# Autodesk Inventor assembly: ASTRA
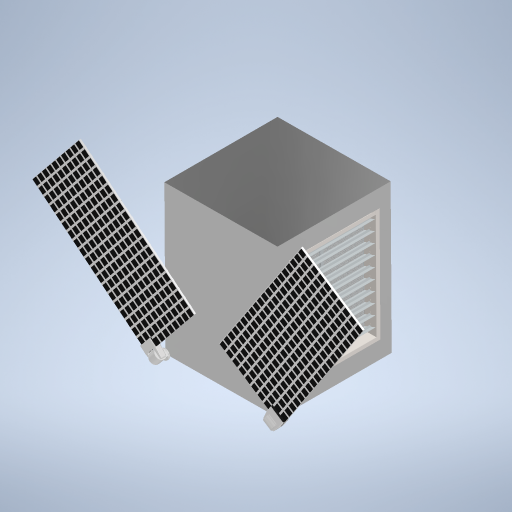
[picture p0: Inventor's stored thumbnail of the model, 512x512]
Saved by Autodesk Inventor 2023.2 (Build 272271030, 271C)
## iProperties
Created: 2023-04-10
Part Number: ASTRA
Document SubType Name: Assembly
Designer: ckeer
Author: ckeer
## Documents named in this file (5)
- F:\Github\School\Prelim\CAD\ASTRA.iam
- F:\Github\School\Prelim\CAD\Solar Panel.ipt
- F:\Github\School\Prelim\CAD\ASTRA_Body.ipt
- F:\Github\School\Prelim\CAD\automatic-louver-1.snapshot.9\Zip Folder\Louver 061516\Louver 061516\Louver 061516.iam
- F:\Github\School\Prelim\CAD\Solar Panel 2.ipt
## Components (5 placed, 4 different names)
1. Solar Panel:1 — Rotational:2
2. ASTRA_Body:1 — Rotational:1, Rotational:2
3. Louver 061516:1 [sub-assembly]
4. Louver 061516:2 [sub-assembly]
5. Solar Panel 2:1 — Rotational:1
## Relationships (2: RevoluteJoint 2)
- Rotational:1 [RevoluteJoint]: ASTRA_Body:1 ↔ Solar Panel 2:1
- Rotational:2 [RevoluteJoint]: Solar Panel:1 ↔ ASTRA_Body:1
